# Autodesk Inventor assembly: Samolot
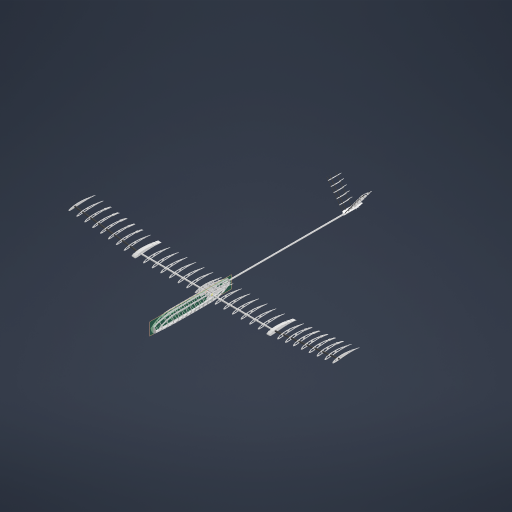
[picture p0: Inventor's stored thumbnail of the model, 512x512]
Saved by Autodesk Inventor 2023 (Build 270158000, 158)
## iProperties
Created: 2023-01-05
Part Number: Samolot
Document SubType Name: Assembly
Designer: szykr
Author: szykr
## Documents named in this file (4)
- D:\Folder Instalacyjny\GitHub Pliki\Solaris\new model\Samolot.iam
- D:\Folder Instalacyjny\GitHub Pliki\Solaris\new model\Skrzydło.iam
- D:\Folder Instalacyjny\GitHub Pliki\Solaris\new model\Tail\Tail.iam
- D:\Folder Instalacyjny\GitHub Pliki\Solaris\new model\nowy kadłub.ipt
## Components (3 placed, 3 different names)
1. Tail:1 [sub-assembly] — Insert:1
2. nowy kadłub:1 — Mate:1, Mate:2, Mate:3, Insert:1
3. Skrzydło:1 [sub-assembly] — Mate:1, Mate:2, Mate:3
## Relationships (4: Mate 3, Insert 1)
- Mate:1: nowy kadłub:1 ↔ Skrzydło:1
- Mate:2: nowy kadłub:1 ↔ Skrzydło:1
- Mate:3: nowy kadłub:1 ↔ Skrzydło:1
- Insert:1 (-40 mm): Tail:1 ↔ nowy kadłub:1
